# Autodesk Inventor assembly: Assembly1
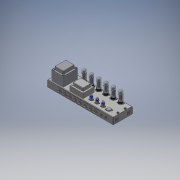
[picture p0: Inventor's stored thumbnail of the model, 180x180]
Saved by Autodesk Inventor 2016 (Build 200138000, 138)
## iProperties
Created: 2015-10-14
Part Number: Assembly1
Document SubType Name: Assembly
Designer: jeremyhale
Author: jeremyhale
## Documents named in this file (35)
- \\psf\Home\Documents\Poorhouse\git\p0001\chassis.iam
- chassis.iam
- \\psf\Home\Documents\Poorhouse\git\p0001\tube socket 8 pin.ipt
- \\psf\Home\Documents\Poorhouse\git\p0001\tube socket 9 pin.ipt
- \\psf\Home\Documents\Poorhouse\git\p0001\xmfr power.ipt
- \\psf\Home\Documents\Poorhouse\git\p0001\xmfr output.ipt
- \\psf\Home\Documents\Inventor\Content Center Files\R2016\en-US\AS 1474(1)\AS 1474 - M3(1).ipt
- \\psf\Home\Documents\Poorhouse\git\p0001\iec320_703W-00_04.ipt
- \\psf\Home\Documents\Inventor\Content Center Files\R2016\en-US\AS 1427(07)\AS 1427 - M3 x 10(6) II.ipt
- \\psf\Home\Documents\Poorhouse\git\p0001\Toggle Large A.ipt
- \\psf\Home\Documents\Poorhouse\git\p0001\AUDIO JACK 2.ipt
- \\psf\Home\Documents\Poorhouse\git\p0001\Bussman fuse holder HKP - 0,25'' X 1,25''.ipt
- \\psf\Home\Documents\Poorhouse\git\p0001\cage nut m6.iam
- \\psf\Home\Documents\Poorhouse\git\p0001\PEC11R-4220F-S0024.ipt
- \\psf\Home\Documents\Inventor\Content Center Files\R2016\en-US\UNI 5590  A\UNI 5590 - A M7.ipt
- \\psf\Home\Documents\Inventor\Content Center Files\R2016\en-US\BS 4320(2)\BS 4320 - M7 (Form B).ipt
- \\psf\Home\Documents\Poorhouse\git\p0001\rotary control.iam
- \\psf\Home\Documents\Poorhouse\git\p0001\Standoff 7mm M2 Wurth 9774070243R.ipt
- \\psf\Home\Documents\Poorhouse\git\p0001\chassis\Design Accelerator\Bolted Connection2.iam
- \\psf\Home\Documents\Poorhouse\git\p0001\chassis\Design Accelerator\Bolted Connection3.iam
- \\psf\Home\Documents\Poorhouse\git\p0001\chassis\Design Accelerator\Bolted Connection4.iam
- \\psf\Home\Documents\Poorhouse\git\p0001\chassis\Design Accelerator\Bolted Connection5.iam
- \\psf\Home\Documents\Poorhouse\git\p0001\chassis\Design Accelerator\Bolted Connection8.iam
- \\psf\Home\Documents\Poorhouse\git\p0001\chassis-weld.iam
- \\psf\Home\Documents\Poorhouse\git\p0001\octal assembly.ipt
- \\psf\Home\Documents\Poorhouse\git\p0001\chassis\Design Accelerator\Bolted Connection6.iam
- \\psf\Home\Documents\Poorhouse\git\p0001\el34 assembly_r1.ipt
- \\psf\Home\Documents\Poorhouse\git\p0001\chassis\Design Accelerator\Bolted Connection7.iam
- \\psf\Home\Documents\Poorhouse\git\p0001\chassis\Design Accelerator\Bolted Connection9.iam
- \\psf\Home\Documents\Poorhouse\git\p0001\Noval socket.ipt
- \\psf\Home\Documents\Poorhouse\git\p0001\12ax7_complete.ipt
- \\psf\Home\Documents\Poorhouse\git\p0001\chassis\Design Accelerator\Bolted Connection10.iam
- \\psf\Home\Documents\Poorhouse\git\p0001\chassis\Design Accelerator\Bolted Connection11.iam
- \\psf\Home\Documents\Poorhouse\git\p0001\chassis\Design Accelerator\Bolted Connection12.iam
- \\psf\Home\Documents\Poorhouse\git\p0001\chassis\Design Accelerator\Bolted Connection13.iam
## Components (206 placed, 25 different names)
1. xmfr power:1 — Mate:55, Flush:4, Flush:5, Mate:68, Mate:69, Mate:70, Mate:71, Mate:72, Mate:73, Mate:74, Mate:75
2. xmfr output:1
3. Bussman fuse holder HKP - 0,25'' X 1,25'':1
4. PowerSwitch
5. chassis-weld:1 [sub-assembly] — Angle:1, Rotational:29, Rotational:30, Insert:43, Angle:2, Rigid:32, Insert:44, Angle:3, Insert:45, Angle:4, Rigid:34, Mate:55, Flush:4, Flush:5
6. big preamp tube socket — Insert:44, Angle:3, Mate:51, Mate:52
7. Bolted Connection:113 [sub-assembly] — Mate:68, Mate:69
8. Bolted Connection:114 [sub-assembly] — Mate:70, Mate:71
9. Bolted Connection:115 [sub-assembly] — Mate:72, Mate:73
10. Bolted Connection:116 [sub-assembly] — Mate:74, Mate:75
11. iec320_703W-00_04:1 — Mate:6, Mate:7
12. AS 1427 Z - Metric M3 x 10:2 — Mate:6, Mate:10
13. AS 1427 Z - Metric M3 x 10:1 — Mate:7, Mate:12
14. AS 1474 - Metric M3:5 — Mate:10
15. AS 1474 - Metric M3:6 — Mate:12
16. cage nut m6:1 [sub-assembly]
17. cage nut m6:2 [sub-assembly]
18. cage nut m6:3 [sub-assembly]
19. cage nut m6:4 [sub-assembly]
20. cage nut m6:5 [sub-assembly]
21. cage nut m6:6 [sub-assembly]
22. cage nut m6:7 [sub-assembly]
23. cage nut m6:8 [sub-assembly]
24. Input Jack
25. AUDIO JACK 2:5
26. Bolted Connection:4 [sub-assembly] — Mate:38
27. Bolted Connection:3 [sub-assembly] — Mate:30
28. Bolted Connection:2 [sub-assembly] — Mate:32
29. Bolted Connection:1 [sub-assembly] — Mate:34
30. Standoff 7mm M2 Wurth 9774070243R:4 — Insert:42, Mate:38
31. Standoff 7mm M2 Wurth 9774070243R:3 — Insert:41, Mate:32
32. Standoff 7mm M2 Wurth 9774070243R:2 — Insert:40, Mate:30
33. Standoff 7mm M2 Wurth 9774070243R:1 — Insert:39, Mate:34
34. rotary control:1 [sub-assembly] — Insert:39, Insert:40, Insert:41, Insert:42, Angle:1, Cylindrical:1, Mate:39, Mate:40
35. BS 4320 Form AB M7 (Form B):1 — Mate:15, Mate:18
36. UNI 5590 A A M7:1 — Mate:17, Mate:18
37. PEC11R-4220F-S0024:1 — Mate:15, Mate:17, Cylindrical:1
38. Bolted Connection:37 [sub-assembly]
39. Bolted Connection:38 [sub-assembly]
40. Bolted Connection:39 [sub-assembly]
41. Bolted Connection:40 [sub-assembly]
42. Standoff 7mm M2 Wurth 9774070243R:5
43. Standoff 7mm M2 Wurth 9774070243R:6
44. Standoff 7mm M2 Wurth 9774070243R:7
45. Standoff 7mm M2 Wurth 9774070243R:8
46. rotary control:2 [sub-assembly]
47. BS 4320 Form AB M7 (Form B):2
48. UNI 5590 A A M7:2
49. PEC11R-4220F-S0024:2
50. Bolted Connection:45 [sub-assembly]
51. Bolted Connection:46 [sub-assembly]
52. Bolted Connection:47 [sub-assembly]
53. Bolted Connection:48 [sub-assembly]
54. Standoff 7mm M2 Wurth 9774070243R:9
55. Standoff 7mm M2 Wurth 9774070243R:10
56. Standoff 7mm M2 Wurth 9774070243R:11
57. Standoff 7mm M2 Wurth 9774070243R:12
58. rotary control:3 [sub-assembly]
59. BS 4320 Form AB M7 (Form B):3
60. UNI 5590 A A M7:3
61. PEC11R-4220F-S0024:3
62. Bolted Connection:53 [sub-assembly]
63. Bolted Connection:54 [sub-assembly]
64. Bolted Connection:55 [sub-assembly]
65. Bolted Connection:56 [sub-assembly]
66. Standoff 7mm M2 Wurth 9774070243R:13
67. Standoff 7mm M2 Wurth 9774070243R:14
68. Standoff 7mm M2 Wurth 9774070243R:15
69. Standoff 7mm M2 Wurth 9774070243R:16
70. rotary control:4 [sub-assembly]
71. BS 4320 Form AB M7 (Form B):4
72. UNI 5590 A A M7:4
73. PEC11R-4220F-S0024:4
74. Bolted Connection:61 [sub-assembly]
75. Bolted Connection:62 [sub-assembly]
76. Bolted Connection:63 [sub-assembly]
77. Bolted Connection:64 [sub-assembly]
78. Standoff 7mm M2 Wurth 9774070243R:17
79. Standoff 7mm M2 Wurth 9774070243R:18
80. Standoff 7mm M2 Wurth 9774070243R:19
81. Standoff 7mm M2 Wurth 9774070243R:20
82. rotary control:5 [sub-assembly]
83. BS 4320 Form AB M7 (Form B):5
84. UNI 5590 A A M7:5
85. PEC11R-4220F-S0024:5
86. Bolted Connection:69 [sub-assembly]
87. Bolted Connection:70 [sub-assembly]
88. Bolted Connection:71 [sub-assembly]
89. Bolted Connection:72 [sub-assembly]
90. Standoff 7mm M2 Wurth 9774070243R:21
91. Standoff 7mm M2 Wurth 9774070243R:22
92. Standoff 7mm M2 Wurth 9774070243R:23
93. Standoff 7mm M2 Wurth 9774070243R:24
94. rotary control:6 [sub-assembly]
95. BS 4320 Form AB M7 (Form B):6
96. UNI 5590 A A M7:6
97. PEC11R-4220F-S0024:6
98. Bolted Connection:77 [sub-assembly]
99. Bolted Connection:78 [sub-assembly]
100. Bolted Connection:79 [sub-assembly]
101. Bolted Connection:80 [sub-assembly]
102. Standoff 7mm M2 Wurth 9774070243R:25
103. Standoff 7mm M2 Wurth 9774070243R:26
104. Standoff 7mm M2 Wurth 9774070243R:27
105. Standoff 7mm M2 Wurth 9774070243R:28
106. rotary control:7 [sub-assembly]
107. BS 4320 Form AB M7 (Form B):7
108. UNI 5590 A A M7:7
109. PEC11R-4220F-S0024:7
110. Bolted Connection:85 [sub-assembly]
111. Bolted Connection:86 [sub-assembly]
112. Bolted Connection:87 [sub-assembly]
113. Bolted Connection:88 [sub-assembly]
114. Standoff 7mm M2 Wurth 9774070243R:29
115. Standoff 7mm M2 Wurth 9774070243R:30
116. Standoff 7mm M2 Wurth 9774070243R:31
117. Standoff 7mm M2 Wurth 9774070243R:32
118. rotary control:8 [sub-assembly]
119. BS 4320 Form AB M7 (Form B):8
120. UNI 5590 A A M7:8
121. PEC11R-4220F-S0024:8
122. AUDIO JACK 2:6 — Rotational:29
123. AUDIO JACK 2:7
124. AUDIO JACK 2:8
125. jack speaker — Rotational:30
126. AUDIO JACK 2:9
127. AUDIO JACK 2:10
128. tube socket 8 pin:1 — Insert:43, Angle:2, Mate:53, Mate:54
129. octal assembly:1 — Rigid:32, Rigid:33
130. el34 assembly_r1:1 — Rigid:33
131. tube socket 8 pin:8
132. octal assembly:2
133. el34 assembly_r1:2
134. tube socket 8 pin:9
135. octal assembly:3
136. el34 assembly_r1:3
137. tube socket 8 pin:10
138. octal assembly:4
139. el34 assembly_r1:4
140. tube socket 8 pin:11
141. octal assembly:5
142. el34 assembly_r1:5
143. tube socket 8 pin:12
144. octal assembly:6
145. el34 assembly_r1:6
146. Bolted Connection:105 [sub-assembly] — Mate:51, Mate:52
147. Bolted Connection:106 [sub-assembly]
148. tube socket 9 pin:1 — Insert:45, Angle:4, Mate:49, Mate:50
149. Noval socket:1 — Rigid:34, Rigid:35
150. 12ax7_complete:1 — Rigid:35
151. tube socket 9 pin:2
152. Noval socket:2
153. 12ax7_complete:2
154. tube socket 9 pin:3
155. Noval socket:3
156. 12ax7_complete:3
157. Bolted Connection:33 [sub-assembly] — Mate:39, Mate:40
158. Bolted Connection:34 [sub-assembly]
159. Bolted Connection:35 [sub-assembly]
160. Bolted Connection:36 [sub-assembly]
161. Bolted Connection:41 [sub-assembly]
162. Bolted Connection:42 [sub-assembly]
163. Bolted Connection:43 [sub-assembly]
164. Bolted Connection:44 [sub-assembly]
165. Bolted Connection:49 [sub-assembly]
166. Bolted Connection:50 [sub-assembly]
167. Bolted Connection:51 [sub-assembly]
168. Bolted Connection:52 [sub-assembly]
169. Bolted Connection:57 [sub-assembly]
170. Bolted Connection:58 [sub-assembly]
171. Bolted Connection:59 [sub-assembly]
172. Bolted Connection:60 [sub-assembly]
173. Bolted Connection:65 [sub-assembly]
174. Bolted Connection:66 [sub-assembly]
175. Bolted Connection:67 [sub-assembly]
176. Bolted Connection:68 [sub-assembly]
177. Bolted Connection:73 [sub-assembly]
178. Bolted Connection:74 [sub-assembly]
179. Bolted Connection:75 [sub-assembly]
180. Bolted Connection:76 [sub-assembly]
181. Bolted Connection:81 [sub-assembly]
182. Bolted Connection:82 [sub-assembly]
183. Bolted Connection:83 [sub-assembly]
184. Bolted Connection:84 [sub-assembly]
185. Bolted Connection:89 [sub-assembly]
186. Bolted Connection:90 [sub-assembly]
187. Bolted Connection:91 [sub-assembly]
188. Bolted Connection:92 [sub-assembly]
189. Bolted Connection:93 [sub-assembly] — Mate:53, Mate:54
190. Bolted Connection:94 [sub-assembly]
191. Bolted Connection:95 [sub-assembly]
192. Bolted Connection:96 [sub-assembly]
193. Bolted Connection:97 [sub-assembly]
194. Bolted Connection:98 [sub-assembly]
195. Bolted Connection:99 [sub-assembly]
196. Bolted Connection:100 [sub-assembly]
197. Bolted Connection:101 [sub-assembly]
198. Bolted Connection:102 [sub-assembly]
199. Bolted Connection:103 [sub-assembly]
200. Bolted Connection:104 [sub-assembly]
201. Bolted Connection:107 [sub-assembly] — Mate:49, Mate:50
202. Bolted Connection:108 [sub-assembly]
203. Bolted Connection:109 [sub-assembly]
204. Bolted Connection:110 [sub-assembly]
205. Bolted Connection:111 [sub-assembly]
206. Bolted Connection:112 [sub-assembly]
## Component patterns: Cage Nuts Top (4 elements), Cage Nuts Right (2 elements), Cage Nuts Left (2 elements), jacks input (2 elements), controls (8 elements), jacks fx (3 elements), jacks speaker (3 elements), big tubes (6 elements), big preamp tube screws (2 elements), small preamp tubes (3 elements), (4 elements, first: Bolted Connection:33), Component Pattern 21:2 (4 elements), Component Pattern 21:3 (4 elements), Component Pattern 21:4 (4 elements), Component Pattern 21:5 (4 elements), Component Pattern 21:6 (4 elements), Component Pattern 21:7 (4 elements), Component Pattern 21:8 (4 elements), big tube socket screws (2 elements), big tube socket screws:2 (2 elements), big tube socket screws:3 (2 elements), big tube socket screws:4 (2 elements), big tube socket screws:5 (2 elements), big tube socket screws:6 (2 elements), small tube screws (2 elements), small tube screws:2 (2 elements), small tube screws:3 (2 elements)
## Relationships (71: Mate 37, WeldJoint 9, RevoluteJoint 8, Insert 7, Flush 5, Angle 4, CylindricalJoint 1)
- [RevoluteJoint]: xmfr output:1 ↔ chassis-weld:1
- [RevoluteJoint]: xmfr output:1 ↔ chassis-weld:1
- [RevoluteJoint]: chassis-weld:1 ↔ iec320_703W-00_04:1
- [RevoluteJoint]: chassis-weld:1 ↔ iec320_703W-00_04:1
- Mate:6: iec320_703W-00_04:1 ↔ AS 1427 Z - Metric M3 x 10:2
- Mate:7: iec320_703W-00_04:1 ↔ AS 1427 Z - Metric M3 x 10:1
- Mate:10: AS 1427 Z - Metric M3 x 10:2 ↔ AS 1474 - Metric M3:5
- [Mate]: chassis-weld:1 ↔ AS 1474 - Metric M3:5
- Mate:12: AS 1427 Z - Metric M3 x 10:1 ↔ AS 1474 - Metric M3:6
- [Mate]: chassis-weld:1 ↔ AS 1474 - Metric M3:6
- [WeldJoint]: Bussman fuse holder HKP - 0,25'' X 1,25'':1 ↔ chassis-weld:1
- [WeldJoint]: PowerSwitch ↔ chassis-weld:1
- [Flush]: chassis-weld:1
- [Flush]: chassis-weld:1
- [Flush]: chassis-weld:1
- [WeldJoint]: chassis-weld:1 ↔ cage nut m6:1
- [WeldJoint]: chassis-weld:1 ↔ cage nut m6:5
- [WeldJoint]: chassis-weld:1 ↔ cage nut m6:7
- Mate:15: BS 4320 Form AB M7 (Form B):1 ↔ PEC11R-4220F-S0024:1
- [Mate]: chassis-weld:1 ↔ BS 4320 Form AB M7 (Form B):1
- Mate:17: UNI 5590 A A M7:1 ↔ PEC11R-4220F-S0024:1
- Mate:18: BS 4320 Form AB M7 (Form B):1 ↔ UNI 5590 A A M7:1
- Insert:39: Standoff 7mm M2 Wurth 9774070243R:1 ↔ rotary control:1
- Insert:40: Standoff 7mm M2 Wurth 9774070243R:2 ↔ rotary control:1
- Insert:41: Standoff 7mm M2 Wurth 9774070243R:3 ↔ rotary control:1
- Insert:42: Standoff 7mm M2 Wurth 9774070243R:4 ↔ rotary control:1
- [Mate]: chassis-weld:1 ↔ Standoff 7mm M2 Wurth 9774070243R:1
- [Mate]: chassis-weld:1 ↔ Standoff 7mm M2 Wurth 9774070243R:4
- Angle:1 (0 deg): chassis-weld:1 ↔ rotary control:1
- Cylindrical:1: rotary control:1 ↔ PEC11R-4220F-S0024:1
- [Mate]: chassis-weld:1 ↔ Bolted Connection:3
- Mate:30: Bolted Connection:3 ↔ Standoff 7mm M2 Wurth 9774070243R:2
- [Mate]: chassis-weld:1 ↔ Bolted Connection:2
- Mate:32: Bolted Connection:2 ↔ Standoff 7mm M2 Wurth 9774070243R:3
- [Mate]: chassis-weld:1 ↔ Bolted Connection:1
- Mate:34: Bolted Connection:1 ↔ Standoff 7mm M2 Wurth 9774070243R:1
- [RevoluteJoint]: chassis-weld:1 ↔ Input Jack
- [RevoluteJoint]: chassis-weld:1 ↔ PEC11R-4220F-S0024:1
- [Mate]: chassis-weld:1 ↔ Bolted Connection:4
- Mate:38: Bolted Connection:4 ↔ Standoff 7mm M2 Wurth 9774070243R:4
- Mate:39: rotary control:1 ↔ Bolted Connection:33
- Mate:40: rotary control:1 ↔ Bolted Connection:33
- Rotational:29 [RevoluteJoint]: chassis-weld:1 ↔ AUDIO JACK 2:6
- Rotational:30 [RevoluteJoint]: chassis-weld:1 ↔ jack speaker
- Insert:43: chassis-weld:1 ↔ tube socket 8 pin:1
- Angle:2 (120 deg): chassis-weld:1 ↔ tube socket 8 pin:1
- Rigid:32 [WeldJoint]: chassis-weld:1 ↔ octal assembly:1
- Rigid:33 [WeldJoint]: octal assembly:1 ↔ el34 assembly_r1:1
- Insert:44: chassis-weld:1 ↔ big preamp tube socket
- Angle:3 (30 deg): chassis-weld:1 ↔ big preamp tube socket
- Insert:45: chassis-weld:1 ↔ tube socket 9 pin:1
- Angle:4 (30 deg): chassis-weld:1 ↔ tube socket 9 pin:1
- Mate:49: tube socket 9 pin:1 ↔ Bolted Connection:107
- Mate:50: tube socket 9 pin:1 ↔ Bolted Connection:107
- Mate:51: big preamp tube socket ↔ Bolted Connection:105
- Mate:52: big preamp tube socket ↔ Bolted Connection:105
- Mate:53: tube socket 8 pin:1 ↔ Bolted Connection:93
- Mate:54: tube socket 8 pin:1 ↔ Bolted Connection:93
- Rigid:34 [WeldJoint]: chassis-weld:1 ↔ Noval socket:1
- Rigid:35 [WeldJoint]: Noval socket:1 ↔ 12ax7_complete:1
- Mate:55: xmfr power:1 ↔ chassis-weld:1
- Flush:4: xmfr power:1 ↔ chassis-weld:1
- Flush:5: xmfr power:1 ↔ chassis-weld:1
- Mate:68: xmfr power:1 ↔ Bolted Connection:113
- Mate:69: xmfr power:1 ↔ Bolted Connection:113
- Mate:70: xmfr power:1 ↔ Bolted Connection:114
- Mate:71: xmfr power:1 ↔ Bolted Connection:114
- Mate:72: xmfr power:1 ↔ Bolted Connection:115
- Mate:73: xmfr power:1 ↔ Bolted Connection:115
- Mate:74: xmfr power:1 ↔ Bolted Connection:116
- Mate:75: xmfr power:1 ↔ Bolted Connection:116
## Named parameters: ControlSpacing = 44.45 mm, tubeAngle = 30 deg
